# Autodesk Inventor assembly: 42146-23
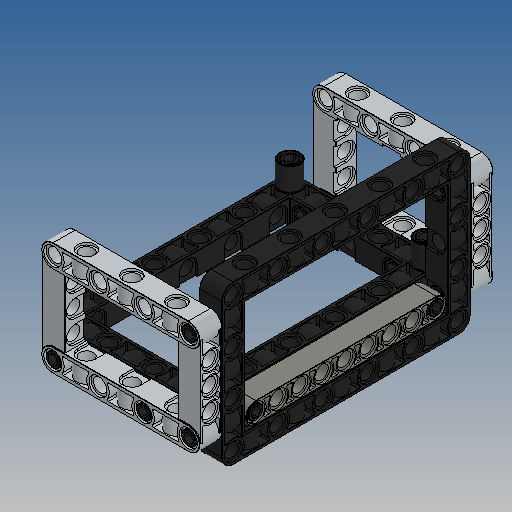
[picture p0: Inventor's stored thumbnail of the model, 512x512]
Saved by Autodesk Inventor 2025 (Build 290162010, 162A)
## iProperties
Created: 2024-11-23
Part Number: 42146-23
Material: Generisch
Document SubType Name: Assembly
Designer: hp.muther
Author: hp.muther
## Documents named in this file (7)
- D:\Inventor\Projekte\Muther\LEGO Technic\LEGO Technik - Raupenkran LR 13000 (42146)\42146-23.iam
- D:\Inventor\Projekte\Muther\LEGO Technic\LEGO Pieces\Rahmen, T-Stücke\39794-Black.ipt
- D:\Inventor\Projekte\Muther\LEGO Technic\LEGO Pieces\Rund\18654-Black.ipt
- D:\Inventor\Projekte\Muther\LEGO Technic\LEGO Pieces\Pin's\2780-Black.ipt
- D:\Inventor\Projekte\Muther\LEGO Technic\LEGO Pieces\Rahmen, T-Stücke\64179-LtBluishGray.ipt
- D:\Inventor\Projekte\Muther\LEGO Technic\LEGO Pieces\Lochbalken\40490-DkBluishGray.ipt
- D:\Inventor\Projekte\Muther\LEGO Technic\LEGO Technik - Raupenkran LR 13000 (42146)\42146_64179_2.ipt
## Components (23 placed, 6 different names)
1. 39794-Black:1 — Einfügen:5, Einfügen:6, Einfügen:7, Einfügen:8, Einfügen:9, Einfügen:10, Einfügen:11, Einfügen:12, Einfügen:17, Einfügen:19, Einfügen:22, Passend:4
2. 18654-Black:1 — Einfügen:1
3. 2780-Black:1 — Einfügen:1, Einfügen:7
4. 18654-Black:2
5. 2780-Black:2 — Einfügen:8
6. 18654-Black:3
7. 2780-Black:3 — Einfügen:6
8. 18654-Black:4
9. 2780-Black:4 — Einfügen:5
10. 2780-Black:5 — Einfügen:11
11. 2780-Black:6 — Einfügen:12, Passend:1
12. 2780-Black:7 — Einfügen:10
13. 2780-Black:8 — Einfügen:9
14. 39794-Black:2 — Einfügen:18
15. 2780-Black:9 — Passend:2
16. 2780-Black:10
17. 2780-Black:11 — Passend:3
18. 2780-Black:12
19. 64179-LtBluishGray:2 — Einfügen:19, Passend:3
20. 40490-DkBluishGray:1 — Einfügen:20, Einfügen:21, Einfügen:22
21. 2780-Black:13 — Einfügen:20, Passend:4
22. 2780-Black:14 — Einfügen:21
23. 42146_64179_2:1 — Einfügen:17, Passend:1, Einfügen:18, Passend:2
## Relationships (26: Insert 22, Mate 4)
- Einfügen:1 [Insert]: 18654-Black:1 ↔ 2780-Black:1
- [Insert]: 18654-Black:2 ↔ 2780-Black:2
- [Insert]: 18654-Black:3 ↔ 2780-Black:3
- [Insert]: 18654-Black:4 ↔ 2780-Black:4
- Einfügen:5 [Insert]: 39794-Black:1 ↔ 2780-Black:4
- Einfügen:6 [Insert]: 39794-Black:1 ↔ 2780-Black:3
- Einfügen:7 [Insert]: 39794-Black:1 ↔ 2780-Black:1
- Einfügen:8 [Insert]: 39794-Black:1 ↔ 2780-Black:2
- Einfügen:9 [Insert]: 39794-Black:1 ↔ 2780-Black:8
- Einfügen:10 [Insert]: 39794-Black:1 ↔ 2780-Black:7
- Einfügen:11 [Insert]: 39794-Black:1 ↔ 2780-Black:5
- Einfügen:12 [Insert]: 39794-Black:1 ↔ 2780-Black:6
- [Insert]: 39794-Black:2 ↔ 2780-Black:12
- [Insert]: 39794-Black:2 ↔ 2780-Black:11
- [Insert]: 39794-Black:2 ↔ 2780-Black:9
- [Insert]: 39794-Black:2 ↔ 2780-Black:10
- Einfügen:17 [Insert]: 39794-Black:1 ↔ 42146_64179_2:1
- Passend:1 [Mate]: 2780-Black:6 ↔ 42146_64179_2:1
- Passend:2 [Mate]: 2780-Black:9 ↔ 42146_64179_2:1
- Einfügen:18 [Insert]: 39794-Black:2 ↔ 42146_64179_2:1
- Einfügen:19 [Insert]: 39794-Black:1 ↔ 64179-LtBluishGray:2
- Passend:3 [Mate]: 2780-Black:11 ↔ 64179-LtBluishGray:2
- Einfügen:20 [Insert]: 40490-DkBluishGray:1 ↔ 2780-Black:13
- Einfügen:21 [Insert]: 40490-DkBluishGray:1 ↔ 2780-Black:14
- Einfügen:22 [Insert]: 39794-Black:1 ↔ 40490-DkBluishGray:1
- Passend:4 [Mate]: 39794-Black:1 ↔ 2780-Black:13
## Named parameters: d1_d0 = 0 mm, d2_d0 = 0 mm, d3_d0 = 0 mm, d12_d8 = 0 mm, d13_d9 = 0 mm, d14_d10 = 0 mm, d15_d11 = 0 mm
